# Autodesk Inventor assembly: x-carriage+chimera
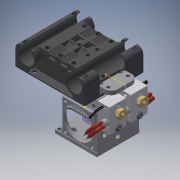
[picture p0: Inventor's stored thumbnail of the model, 180x180]
Saved by Autodesk Inventor 2019 (Build 230136000, 136)
## iProperties
Created: 2020-01-18
Part Number: x-carriage+chimera
Material: Generisch
Document SubType Name: Assembly
Designer: marc
Author: marc
## Documents named in this file (6)
- C:\Users\marc\Google Drive\Projekte\3D Drucker\brezzlicator\1. Printed Parts\3. Modified by marc\x-carriage+chimera.iam
- C:\Users\marc\Google Drive\Projekte\3D Drucker\brezzlicator\1. Printed Parts\3. Modified by marc\inventor\x_carriage_aio_base.ipt
- C:\Users\marc\Downloads\CyclopPlus Assembly.iam
- C:\Users\marc\Downloads\Aqua + Heatsink.iam
- C:\Users\marc\Google Drive\Projekte\3D Drucker\brezzlicator\1. Printed Parts\3. Modified by marc\dual_fan_adapter.ipt
- C:\Users\marc\Google Drive\Projekte\3D Drucker\brezzlicator\1. Printed Parts\3. Modified by marc\inventor\x_carriage_aio_ir_probe.ipt
## Components (5 placed, 5 different names)
1. x_carriage_aio_base:1 — Drehbar:1, Drehbar:3
2. CyclopPlus Assembly:1 [sub-assembly] — Zylindrisch:1, Drehbar:1, Drehbar:2
3. Aqua + Heatsink:1 [sub-assembly] — Zylindrisch:1
4. dual_fan_adapter:1 — Drehbar:2
5. x_carriage_aio_ir_probe:1 — Drehbar:3
## Relationships (4: RevoluteJoint 3, CylindricalJoint 1)
- Zylindrisch:1 [CylindricalJoint]: CyclopPlus Assembly:1 ↔ Aqua + Heatsink:1
- Drehbar:1 [RevoluteJoint]: x_carriage_aio_base:1 ↔ CyclopPlus Assembly:1
- Drehbar:2 [RevoluteJoint]: CyclopPlus Assembly:1 ↔ dual_fan_adapter:1
- Drehbar:3 [RevoluteJoint]: x_carriage_aio_base:1 ↔ x_carriage_aio_ir_probe:1
